# Autodesk Inventor assembly: base
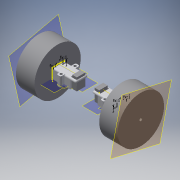
[picture p0: Inventor's stored thumbnail of the model, 180x180]
Saved by Autodesk Inventor 2018 (Build 220112000, 112)
## iProperties
Created: 2017-09-29
Part Number: base
Document SubType Name: Assembly
Designer: fabre
d0: 0,000 mm
d1: 0,000 mm
base_L: 85,000 mm
wheel_shaft_percentage: 0,315 ul
pico_dist: 15,000 mm
laser: 0,200 mm
thick: 4,990 mm
d11: 0,000 mm
d12: -89,000 mm
d13: 0,000 mm
base_fix_holes_dist: 7,000 mm
extra_wood: 2,495 mm
pen_d: 20,000 mm
fente_l: 9,801 mm
nb_fentes: 4,000 ul
male_l: 10,201 mm
batt_hole_l: 35,000 mm
finger_l: 17,000 mm
chepeau_L: 89,990 mm
vis_moteur_d: 2,800 mm
cale_d: 5,000 mm
charniere_epaisseur_axe: 2,600 mm
charniere_trou_d: 2,500 mm
charniere_distance_trou: 8,250 mm
charniere_ecart: 17,200 mm
charniere_L: 24,100 mm
inclinaison: 10,00 deg
tete_hole_margin: 0,100 mm
chanfrein: 1,000 mm
charniere_edge2hole: 7,800 mm
Author: fabre
## Documents named in this file (2)
- C:\Users\rfabre\Desktop\cubi\mechanics\base.iam
- C:\Users\rfabre\Desktop\cubi\mechanics\motor_block.iam
## Components (2 placed, 1 different names)
1. motor_block:1 [sub-assembly] — Flush:1, Flush:2, Mate:1, Mate:2, Mate:3
2. motor_block:2 [sub-assembly] — Flush:1, Mate:1, Mate:2
## Relationships (5: Mate 3, Flush 2)
- Flush:1: motor_block:1 ↔ motor_block:2
- Flush:2: motor_block:1
- Mate:1: motor_block:1 ↔ motor_block:2
- Mate:2 (-89 mm): motor_block:1 ↔ motor_block:2
- Mate:3: motor_block:1
## Named parameters: base_L = 85 mm, wheel_shaft_percentage = 0.315, pico_dist = 15 mm, laser = 0.2 mm, thick = 4.99 mm, base_fix_holes_dist = 7 mm, extra_wood = 2.495 mm, pen_d = 20 mm, fente_l = 4.79 mm, nb_fentes = 4, fente_L = 9.80125 mm, male_l = 5.19 mm, male_L = 10.20125 mm, batt_hole_l = 15 mm, batt_hole_L = 35 mm, finger_l = 10 mm, finger_L = 17 mm, chepeau_L = 89.99 mm, vis_moteur_d = 2.8 mm, cale_d = 5 mm, charniere_epaisseur_axe = 2.6 mm, charniere_trou_d = 2.5 mm, charniere_distance_trou = 8.25 mm, charniere_ecart = 17.2 mm, charniere_L = 24.1 mm, tete_hole_margin = 0.1 mm, inclinaison = 10 deg, chanfrein = 1 mm, charniere_edge2hole = 7.8 mm
